# Autodesk Inventor assembly: Rubiks Cube Solver
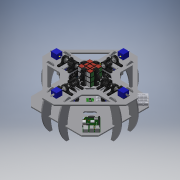
[picture p0: Inventor's stored thumbnail of the model, 180x180]
Saved by Autodesk Inventor 2017 (Build 210142000, 142)
## iProperties
Created: 2018-11-23
Part Number: Rubiks Cube Solver
Document SubType Name: Assembly
Designer: Eric the Great
Author: Eric the Great
## Documents named in this file (19)
- C:\Users\Eric the Great\Documents\Cornell University\ECE 5725\Final Project\CAD\Rubiks Cube Solver.iam
- C:\Users\Eric the Great\Documents\Cornell University\ECE 5725\Final Project\CAD\Nema 17.ipt
- C:\Users\Eric the Great\Documents\Cornell University\ECE 5725\Final Project\CAD\Solenoid.ipt
- C:\Users\Eric the Great\Documents\Cornell University\ECE 5725\Final Project\CAD\8mmx22mm bearing.ipt
- C:\Users\Eric the Great\Documents\Cornell University\ECE 5725\Final Project\CAD\Claw.ipt
- C:\Users\Eric the Great\Documents\Cornell University\ECE 5725\Final Project\CAD\solenoid piston.ipt
- C:\Users\Eric the Great\Documents\Cornell University\ECE 5725\Final Project\CAD\bearing block.ipt
- C:\Users\Eric the Great\Documents\Cornell University\ECE 5725\Final Project\CAD\stepper mount.ipt
- C:\Users\Eric the Great\Documents\Cornell University\ECE 5725\Final Project\CAD\axle.ipt
- C:\Users\Eric the Great\Documents\Cornell University\ECE 5725\Final Project\Rubiks Cube Solver\Design Accelerator\big gear.ipt
- C:\Users\Eric the Great\Documents\Cornell University\ECE 5725\Final Project\Rubiks Cube Solver\Design Accelerator\little gear.ipt
- C:\Users\Eric the Great\Documents\Cornell University\ECE 5725\Final Project\CAD\Rubik's Chassis.iam
- C:\Users\Eric the Great\Documents\Cornell University\ECE 5725\Final Project\CAD\riser1.7mm.ipt
- C:\Users\Eric the Great\Documents\Cornell University\ECE 5725\Final Project\CAD\RspCameraMia.ipt
- C:\Users\Eric the Great\Documents\Cornell University\ECE 5725\Final Project\CAD\camera strand.ipt
- C:\Users\Eric the Great\Documents\Cornell University\ECE 5725\Final Project\CAD\Rpi3Bplus.ipt
- C:\Users\Eric the Great\Documents\Cornell University\ECE 5725\Final Project\CAD\BREADBOARD 60 ROW.ipt
- C:\Users\Eric the Great\Documents\Cornell University\ECE 5725\Final Project\CAD\relay.ipt
- C:\Users\Eric the Great\Documents\Cornell University\ECE 5725\Final Project\CAD\3x3 Rubik's Cube.ipt
## Components (56 placed, 18 different names)
1. Rubik's Chassis:1 [sub-assembly] — Mate:10, Mate:11, Mate:12, Mate:13, Mate:21, Flush:2, Flush:3, Mate:31, Mate:32, Flush:6, Mate:33, Mate:34, Flush:7, Mate:35, Flush:8, Mate:36, Mate:37
2. 3x3 Rubik's Cube:1 — Mate:36, Mate:37, Mate:39
3. riser1.7mm:1 — Mate:19, Mate:20, Flush:1
4. RspCameraMia:1 — Mate:30, Flush:4, Mate:32, Flush:5
5. camera strand:1 — Mate:30, Flush:4, Mate:31, Flush:5
6. Rpi3Bplus:1 — Flush:6, Mate:33
7. BREADBOARD 60 ROW:1 — Mate:34, Flush:7
8. relay:1 — Mate:35, Flush:8
9. Claw:1 — Mate:14, Mate:15
10. bearing block:3 — Mate:3, Mate:8, Mate:10, Mate:12, Mate:38
11. Spur Gear1:1 — Mate:25, Mate:28
12. bearing block:1 — Mate:3, Mate:9, Mate:11, Mate:13, Mate:22
13. solenoid piston:1 — Mate:16, Mate:29
14. Solenoid:1 — Mate:16, Mate:17, Mate:18, Mate:19, Mate:20, Flush:1, Flush:3
15. Spur Gear2:1 — Mate:26, Mate:27
16. stepper mount:1 — Mate:21, Mate:22, Flush:2, Mate:23, Mate:24, Mate:27
17. Nema 17:1 — Mate:18, Mate:23, Mate:24, Mate:26
18. 8mmx22mm bearing:4 — Mate:6, Mate:7, Mate:8, Mate:38
19. 8mmx22mm bearing:3 — Mate:6, Mate:9
20. axle:1 — Mate:7, Mate:14, Mate:15, Mate:17, Mate:25, Mate:28, Mate:29, Mate:39
21. Claw:2
22. bearing block:4
23. Spur Gear1:2
24. bearing block:5
25. solenoid piston:2
26. Solenoid:2
27. Spur Gear2:2
28. stepper mount:2
29. Nema 17:2
30. 8mmx22mm bearing:5
31. 8mmx22mm bearing:6
32. axle:2
33. Claw:3
34. bearing block:6
35. Spur Gear1:3
36. bearing block:7
37. solenoid piston:3
38. Solenoid:3
39. Spur Gear2:3
40. stepper mount:3
41. Nema 17:3
42. 8mmx22mm bearing:7
43. 8mmx22mm bearing:8
44. axle:3
45. Claw:4
46. bearing block:8
47. Spur Gear1:4
48. bearing block:9
49. solenoid piston:4
50. Solenoid:4
51. Spur Gear2:4
52. stepper mount:4
53. Nema 17:4
54. 8mmx22mm bearing:9
55. 8mmx22mm bearing:10
56. axle:4
## Component patterns: (4 elements, first: Claw:1 + bearing block:3 + Spur Gear1:1 + bearing block:1 + solenoid piston:1 + Solenoid:1 + Spur Gear2:1 + stepper mount:1 + Nema 17:1 + 8mmx22mm bearing:4 + 8mmx22mm bearing:3 + axle:1)
## Relationships (43: Mate 35, Flush 8)
- Mate:3: bearing block:3 ↔ bearing block:1
- Mate:6: 8mmx22mm bearing:4 ↔ 8mmx22mm bearing:3
- Mate:7: 8mmx22mm bearing:4 ↔ axle:1
- Mate:8: bearing block:3 ↔ 8mmx22mm bearing:4
- Mate:9: bearing block:1 ↔ 8mmx22mm bearing:3
- Mate:10: Rubik's Chassis:1 ↔ bearing block:3
- Mate:11: Rubik's Chassis:1 ↔ bearing block:1
- Mate:12: Rubik's Chassis:1 ↔ bearing block:3
- Mate:13: Rubik's Chassis:1 ↔ bearing block:1
- Mate:14: Claw:1 ↔ axle:1
- Mate:15: Claw:1 ↔ axle:1
- Mate:16: solenoid piston:1 ↔ Solenoid:1
- Mate:17: Solenoid:1 ↔ axle:1
- Mate:18: Solenoid:1 ↔ Nema 17:1
- Mate:19: riser1.7mm:1 ↔ Solenoid:1
- Mate:20: riser1.7mm:1 ↔ Solenoid:1
- Flush:1: riser1.7mm:1 ↔ Solenoid:1
- Mate:21: Rubik's Chassis:1 ↔ stepper mount:1
- Mate:22: bearing block:1 ↔ stepper mount:1
- Flush:2: Rubik's Chassis:1 ↔ stepper mount:1
- Mate:23: stepper mount:1 ↔ Nema 17:1
- Mate:24: stepper mount:1 ↔ Nema 17:1
- Mate:25: Spur Gear1:1 ↔ axle:1
- Mate:26: Spur Gear2:1 ↔ Nema 17:1
- Mate:27 (4 mm): Spur Gear2:1 ↔ stepper mount:1
- Mate:28: Spur Gear1:1 ↔ axle:1
- Mate:29: solenoid piston:1 ↔ axle:1
- Flush:3 (25 mm): Rubik's Chassis:1 ↔ Solenoid:1
- Mate:30: RspCameraMia:1 ↔ camera strand:1
- Flush:4 (2 mm): RspCameraMia:1 ↔ camera strand:1
- Mate:31: Rubik's Chassis:1 ↔ camera strand:1
- Mate:32: Rubik's Chassis:1 ↔ RspCameraMia:1
- Flush:5: RspCameraMia:1 ↔ camera strand:1
- Flush:6 (15 mm): Rubik's Chassis:1 ↔ Rpi3Bplus:1
- Mate:33: Rubik's Chassis:1 ↔ Rpi3Bplus:1
- Mate:34: Rubik's Chassis:1 ↔ BREADBOARD 60 ROW:1
- Flush:7 (3 mm): Rubik's Chassis:1 ↔ BREADBOARD 60 ROW:1
- Mate:35: Rubik's Chassis:1 ↔ relay:1
- Flush:8 (25 mm): Rubik's Chassis:1 ↔ relay:1
- Mate:36: Rubik's Chassis:1 ↔ 3x3 Rubik's Cube:1
- Mate:37: Rubik's Chassis:1 ↔ 3x3 Rubik's Cube:1
- Mate:38: bearing block:3 ↔ 8mmx22mm bearing:4
- Mate:39: 3x3 Rubik's Cube:1 ↔ axle:1
